# Autodesk Inventor assembly: axle_gear
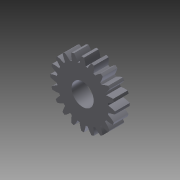
[picture p0: Inventor's stored thumbnail of the model, 180x180]
Saved by Autodesk Inventor 2015 (Build 190159000, 159)
## iProperties
Created: 2015-06-18
Part Number: axle_gear
Document SubType Name: Assembly
Designer: Abhishyant
Author: Abhishyant
## Documents named in this file (4)
- D:\Projects\Personal\BroBot\3D Model\axle_gear.iam
- D:\Projects\Personal\BroBot\3D Model\axle_gear\Design Accelerator\Spur Gears1.iam
- D:\Projects\Personal\BroBot\3D Model\axle_gear\Design Accelerator\Spur Gears6.iam
- D:\Projects\Personal\BroBot\3D Model\gear_axle_hole_maker.ipt
## Components (3 placed, 2 different names)
1. Spur Gears:1 [sub-assembly]
2. gear_axle_hole_maker:1 — Mate:1
3. Spur Gears:2 [sub-assembly] — Mate:1
## Relationships (1: Mate 1)
- Mate:1: gear_axle_hole_maker:1 ↔ Spur Gears:2
